# Autodesk Inventor assembly: (FINAL) CORNER RH
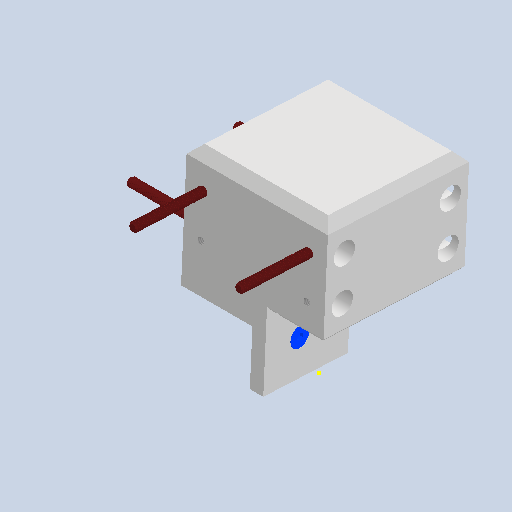
[picture p0: Inventor's stored thumbnail of the model, 512x512]
Saved by Autodesk Inventor 2022 (Build 260153000, 153)
## iProperties
Created: 2022-11-16
Part Number: (FINAL) CORNER RH
Document SubType Name: Assembly
Designer: matia
Author: matia
## Documents named in this file (4)
- C:\Users\matia\Desktop\(V2) FULL ASSEMBLY\(FINAL) CORNER RH.iam
- C:\Users\matia\Desktop\(V2) FULL ASSEMBLY\(FINAL)CORNER.ipt
- C:\Users\matia\Desktop\(V2) FULL ASSEMBLY\91253A139_Black-Oxide Alloy Steel Hex Drive Flat Head Screw_corners.ipt
- C:\Users\matia\Desktop\(V2) FULL ASSEMBLY\91263A139_Zinc-Plated Alloy Steel Hex Drive Flat Head Screw(CORNER2BOARD).ipt
## Components (7 placed, 3 different names)
1. (FINAL)CORNER:1 — Mate:1, Mate:2, Mate:3, Mate:4, Mate:5, Mate:6, Mate:7, Mate:8, Mate:9, Mate:10, Mate:11, Mate:12
2. 91253A139_Black-Oxide Alloy Steel Hex Drive Flat Head Screw_corners:1 — Mate:1, Mate:3
3. 91253A139_Black-Oxide Alloy Steel Hex Drive Flat Head Screw_corners:2 — Mate:5, Mate:8
4. 91253A139_Black-Oxide Alloy Steel Hex Drive Flat Head Screw_corners:3 — Mate:6, Mate:7
5. 91253A139_Black-Oxide Alloy Steel Hex Drive Flat Head Screw_corners:4 — Mate:2, Mate:4
6. 91263A139_Zinc-Plated Alloy Steel Hex Drive Flat Head Screw(CORNER2BOARD):1 — Mate:9, Mate:10
7. 91263A139_Zinc-Plated Alloy Steel Hex Drive Flat Head Screw(CORNER2BOARD):2 — Mate:11, Mate:12
## Relationships (12: Mate 12)
- Mate:1: (FINAL)CORNER:1 ↔ 91253A139_Black-Oxide Alloy Steel Hex Drive Flat Head Screw_corners:1
- Mate:2: (FINAL)CORNER:1 ↔ 91253A139_Black-Oxide Alloy Steel Hex Drive Flat Head Screw_corners:4
- Mate:3: (FINAL)CORNER:1 ↔ 91253A139_Black-Oxide Alloy Steel Hex Drive Flat Head Screw_corners:1
- Mate:4: (FINAL)CORNER:1 ↔ 91253A139_Black-Oxide Alloy Steel Hex Drive Flat Head Screw_corners:4
- Mate:5: (FINAL)CORNER:1 ↔ 91253A139_Black-Oxide Alloy Steel Hex Drive Flat Head Screw_corners:2
- Mate:6: (FINAL)CORNER:1 ↔ 91253A139_Black-Oxide Alloy Steel Hex Drive Flat Head Screw_corners:3
- Mate:7: (FINAL)CORNER:1 ↔ 91253A139_Black-Oxide Alloy Steel Hex Drive Flat Head Screw_corners:3
- Mate:8: (FINAL)CORNER:1 ↔ 91253A139_Black-Oxide Alloy Steel Hex Drive Flat Head Screw_corners:2
- Mate:9: (FINAL)CORNER:1 ↔ 91263A139_Zinc-Plated Alloy Steel Hex Drive Flat Head Screw(CORNER2BOARD):1
- Mate:10: (FINAL)CORNER:1 ↔ 91263A139_Zinc-Plated Alloy Steel Hex Drive Flat Head Screw(CORNER2BOARD):1
- Mate:11: (FINAL)CORNER:1 ↔ 91263A139_Zinc-Plated Alloy Steel Hex Drive Flat Head Screw(CORNER2BOARD):2
- Mate:12: (FINAL)CORNER:1 ↔ 91263A139_Zinc-Plated Alloy Steel Hex Drive Flat Head Screw(CORNER2BOARD):2
